# Autodesk Inventor assembly: Peristaltic pump with extension
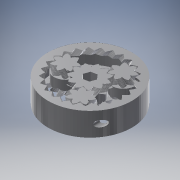
[picture p0: Inventor's stored thumbnail of the model, 180x180]
Saved by Autodesk Inventor 2017 (Build 210142000, 142)
## iProperties
Created: 2016-11-08
Part Number: Peristaltic pump with extension
Document SubType Name: Assembly
Designer: Camilo
Author: Camilo
## Documents named in this file (2)
- Z:\Github\AgingTests\3D parts\Peristaltic pump adapter\Peristaltic pump with extension.iam
- Z:\Github\AgingTests\3D parts\Peristaltic pump adapter\Peristaltic Pump.ipt
## Components (1 placed, 1 different names)
1. Peristaltic Pump:1 — Mate:1, Mate:2, Flush:1
## Relationships (3: Mate 2, Flush 1)
- Mate:1: Peristaltic Pump:1
- Mate:2: Peristaltic Pump:1
- Flush:1: Peristaltic Pump:1
